# Autodesk Inventor assembly: chassis_2-02
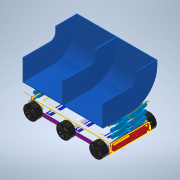
[picture p0: Inventor's stored thumbnail of the model, 180x180]
Saved by Autodesk Inventor 2022 (Build 260153000, 153)
## iProperties
Created: 2023-03-24
Part Number: chassis_2-02
Document SubType Name: Assembly
Designer: Johnny Jou
Author: Johnny Jou
## Documents named in this file (24)
- C:\Users\JOU\Desktop\git\Areo_Rider_Cabin\car\chassis_2.iam
- C:\Users\JOU\Desktop\git\Areo_Rider_Cabin\car\chassis_1_1.ipt
- C:\Users\JOU\Desktop\git\Areo_Rider_Cabin\car\chassis_1_2.ipt
- C:\Users\JOU\Desktop\git\Areo_Rider_Cabin\car\wheel.ipt
- C:\Users\JOU\Desktop\git\Areo_Rider_Cabin\car\wheel_base_cover.ipt
- C:\Users\JOU\Desktop\git\Areo_Rider_Cabin\car\bearing.iam
- C:\Users\JOU\Desktop\git\Areo_Rider_Cabin\car\axle 4_20.ipt
- C:\Users\JOU\Desktop\git\Areo_Rider_Cabin\car\Coupling.ipt
- C:\Users\JOU\Desktop\git\Areo_Rider_Cabin\car\chassis_1_1\chassis_1_1-01.ipt
- C:\Users\JOU\Desktop\git\Areo_Rider_Cabin\Expansion\gasket.ipt
- C:\Users\JOU\Desktop\git\Areo_Rider_Cabin\Expansion\link_2022.ipt
- C:\Users\JOU\Desktop\git\Areo_Rider_Cabin\Expansion\rod_2.ipt
- C:\Users\JOU\Desktop\git\Areo_Rider_Cabin\car\chassis_1_1\chassis_1_1-02.ipt
- C:\Users\JOU\Desktop\git\Areo_Rider_Cabin\car\外抓檔\25GA370.ipt
- C:\Users\JOU\Desktop\git\Areo_Rider_Cabin\Expansion\rod_3.ipt
- C:\Users\JOU\Desktop\git\Areo_Rider_Cabin\car\chassis_1_3.ipt
- C:\Users\JOU\Desktop\git\Areo_Rider_Cabin\car\chassis_1_4.ipt
- C:\Users\JOU\Desktop\git\Areo_Rider_Cabin\car\chassis_1_2_up.ipt
- C:\Users\JOU\Desktop\git\Areo_Rider_Cabin\Airfoil & Nuzzle\nuzzle\nuzzle_v2_0327.ipt
- C:\Users\Johnny Jou\Documents\GitHub\Areo_Rider_Cabin\car\chassis_2\AIP\FEA\eaz3jbjy8.fins
- C:\Users\Johnny Jou\Documents\GitHub\Areo_Rider_Cabin\car\chassis_2\AIP\FEA\eaz3jbjy8.fsat
- C:\Users\Johnny Jou\Documents\GitHub\Areo_Rider_Cabin\car\chassis_2\AIP\FEA\eaz3jbjy8.ftes
- C:\Users\Johnny Jou\Documents\GitHub\Areo_Rider_Cabin\car\chassis_2\AIP\FEA\eaz3jbjy8.fwiz
- C:\Users\Johnny Jou\Documents\GitHub\Areo_Rider_Cabin\car\chassis_2\AIP\FEA\eaz3jbk9s.fmsh
## Components (61 placed, 17 different names)
1. chassis_1_1-02:1 — 貼合:1, 齊平:1, 貼合:2, 齊平:2, 貼合:4, 貼合:5, 貼合:8, 貼合:9, 貼合:10, 貼合:14, 貼合:28, 貼合:29, 貼合:30, 貼合:31, 貼合:39, 貼合:40, 貼合:41, 齊平:12, 貼合:102, 齊平:13, 貼合:103, 貼合:104, 貼合:105, 齊平:14, 貼合:106, 齊平:15, 貼合:110, 貼合:111
2. chassis_1_2:1 — 貼合:1, 齊平:1, 貼合:2, 貼合:62, 角度:1, 相切:2, 貼合:96, 貼合:97, 齊平:17
3. chassis_1_2:2 — 齊平:2, 貼合:4, 貼合:5, 貼合:6, 貼合:7, 齊平:3, 相切:1, 貼合:93, 貼合:95, 貼合:109
4. chassis_1_1-01:2 — 貼合:6, 貼合:7, 齊平:3, 貼合:18, 貼合:19, 貼合:20, 貼合:21, 貼合:56, 貼合:57, 貼合:58, 貼合:59, 貼合:60, 貼合:61, 齊平:11, 貼合:107, 貼合:108
5. 25GA370:1 — 貼合:8, 貼合:9, 貼合:10, 貼合:11
6. Coupling:1 — 貼合:11, 貼合:12, 貼合:13, 貼合:14
7. wheel:1 — 貼合:12, 貼合:13
8. 25GA370:2 — 貼合:18, 貼合:20, 貼合:21
9. Coupling:2 — 貼合:19
10. wheel:2
11. Coupling:3 — 貼合:27, 貼合:28
12. wheel:3
13. 軸承:1 [sub-assembly] — 貼合:24, 貼合:25, 貼合:26, 齊平:4
14. wheel_base_cover:1 — 貼合:24, 貼合:25, 貼合:30, 貼合:31
15. axle 4_20:1 — 貼合:26, 齊平:4, 貼合:27, 貼合:29
16. Coupling:4 — 貼合:38
17. wheel:4
18. 軸承:2 [sub-assembly]
19. wheel_base_cover:2 — 貼合:38, 貼合:39, 貼合:40, 貼合:41
20. axle 4_20:2
21. Coupling:5
22. wheel:5
23. 軸承:3 [sub-assembly]
24. wheel_base_cover:3 — 貼合:56, 貼合:57, 貼合:58
25. axle 4_20:3
26. Coupling:6
27. wheel:6 — 齊平:16
28. 軸承:4 [sub-assembly]
29. wheel_base_cover:4 — 貼合:59, 貼合:60, 貼合:61
30. axle 4_20:4
31. rod_2:1 — 貼合:62, 角度:1, 貼合:63, 貼合:64, 貼合:65, 貼合:66, 貼合:94, 貼合:98
32. 軸承:5 [sub-assembly] — 貼合:63, 貼合:64, 相切:1
33. 軸承:6 [sub-assembly] — 貼合:65, 貼合:66, 相切:2
34. link_2022:1 — 貼合:67, up_and_down, 貼合:70, 貼合:71, 貼合:75, 貼合:94, 插入:3, 齊平:9, 貼合:100
35. link_2022:2 — 貼合:67, up_and_down, 貼合:70, 貼合:76, 貼合:91, 貼合:92, 貼合:93
36. link_2022:3 — 貼合:72, 貼合:76, 貼合:78, 齊平:8, 貼合:99
37. link_2022:4 — 貼合:71, 貼合:72, 貼合:73, 貼合:75, 貼合:77
38. link_2022:5 — 貼合:73, 貼合:74, 貼合:77, 齊平:10, 貼合:101, 插入:6
39. link_2022:6 — 貼合:74, 貼合:78, 貼合:112
40. link_2022:7 — 貼合:96, 貼合:97, 插入:2
41. link_2022:8 — 貼合:98, 插入:1
42. link_2022:9
43. link_2022:10
44. link_2022:11 — 貼合:113
45. link_2022:12 — 插入:4
46. gasket:1 — 貼合:91, 貼合:92, 貼合:95
47. gasket:2 — 插入:1
48. gasket:3 — 插入:2
49. gasket:4 — 插入:3
50. rod_3:1 — 齊平:8, 貼合:99
51. rod_3:2 — 齊平:9, 貼合:100
52. rod_3:3 — 齊平:10, 貼合:101
53. chassis_1_3:1 — 齊平:11, 齊平:12, 貼合:102
54. chassis_1_3:2 — 齊平:15, 貼合:110, 貼合:111
55. chassis_1_3:3 — 齊平:13, 貼合:103, 貼合:104
56. chassis_1_3:4 — 貼合:105, 齊平:14, 貼合:106
57. chassis_1_4:1 — 貼合:107, 貼合:108, 貼合:109
58. chassis_1_2_up:1 — 插入:5, 貼合:112, 貼合:114
59. chassis_1_2_up:2 — 插入:4, 貼合:113
60. gasket:5 — 插入:5, 插入:6
61. nuzzle_v2_0327:1 — 貼合:114, 齊平:16, 齊平:17
## Relationships (145: Mate 113, Flush 17, Angle 7, Insert 6, Tangent 2)
- 貼合:1 [Mate]: chassis_1_1-02:1 ↔ chassis_1_2:1
- 齊平:1 [Flush]: chassis_1_1-02:1 ↔ chassis_1_2:1
- 貼合:2 [Mate]: chassis_1_1-02:1 ↔ chassis_1_2:1
- 齊平:2 [Flush]: chassis_1_1-02:1 ↔ chassis_1_2:2
- 貼合:4 [Mate]: chassis_1_1-02:1 ↔ chassis_1_2:2
- 貼合:5 [Mate]: chassis_1_1-02:1 ↔ chassis_1_2:2
- 貼合:6 [Mate]: chassis_1_2:2 ↔ chassis_1_1-01:2
- 貼合:7 [Mate]: chassis_1_2:2 ↔ chassis_1_1-01:2
- 齊平:3 [Flush]: chassis_1_2:2 ↔ chassis_1_1-01:2
- 貼合:8 [Mate]: chassis_1_1-02:1 ↔ 25GA370:1
- 貼合:9 [Mate]: chassis_1_1-02:1 ↔ 25GA370:1
- 貼合:10 [Mate]: chassis_1_1-02:1 ↔ 25GA370:1
- 貼合:11 [Mate]: 25GA370:1 ↔ Coupling:1
- 貼合:12 [Mate]: Coupling:1 ↔ wheel:1
- 貼合:13 [Mate]: Coupling:1 ↔ wheel:1
- 貼合:14 [Mate] (3 mm): chassis_1_1-02:1 ↔ Coupling:1
- [Mate]: 25GA370:2 ↔ Coupling:2
- [Mate]: Coupling:2 ↔ wheel:2
- [Mate]: Coupling:2 ↔ wheel:2
- 貼合:18 [Mate]: chassis_1_1-01:2 ↔ 25GA370:2
- 貼合:19 [Mate] (3 mm): chassis_1_1-01:2 ↔ Coupling:2
- 貼合:20 [Mate]: chassis_1_1-01:2 ↔ 25GA370:2
- 貼合:21 [Mate]: chassis_1_1-01:2 ↔ 25GA370:2
- [Mate]: Coupling:3 ↔ wheel:3
- [Mate]: Coupling:3 ↔ wheel:3
- 貼合:24 [Mate]: 軸承:1 ↔ wheel_base_cover:1
- 貼合:25 [Mate]: 軸承:1 ↔ wheel_base_cover:1
- 貼合:26 [Mate]: 軸承:1 ↔ axle 4_20:1
- 齊平:4 [Flush]: 軸承:1 ↔ axle 4_20:1
- 貼合:27 [Mate]: Coupling:3 ↔ axle 4_20:1
- 貼合:28 [Mate] (3 mm): chassis_1_1-02:1 ↔ Coupling:3
- 貼合:29 [Mate]: chassis_1_1-02:1 ↔ axle 4_20:1
- 貼合:30 [Mate]: chassis_1_1-02:1 ↔ wheel_base_cover:1
- 貼合:31 [Mate]: chassis_1_1-02:1 ↔ wheel_base_cover:1
- [Mate]: Coupling:4 ↔ wheel:4
- [Mate]: Coupling:4 ↔ wheel:4
- [Mate]: 軸承:2 ↔ wheel_base_cover:2
- [Mate]: 軸承:2 ↔ wheel_base_cover:2
- [Mate]: 軸承:2 ↔ axle 4_20:2
- [Flush]: 軸承:2 ↔ axle 4_20:2
- [Mate]: Coupling:4 ↔ axle 4_20:2
- 貼合:38 [Mate] (6 mm): Coupling:4 ↔ wheel_base_cover:2
- 貼合:39 [Mate]: chassis_1_1-02:1 ↔ wheel_base_cover:2
- 貼合:40 [Mate]: chassis_1_1-02:1 ↔ wheel_base_cover:2
- 貼合:41 [Mate]: chassis_1_1-02:1 ↔ wheel_base_cover:2
- [Mate]: Coupling:5 ↔ wheel:5
- [Mate]: Coupling:5 ↔ wheel:5
- [Mate]: 軸承:3 ↔ wheel_base_cover:3
- [Mate]: 軸承:3 ↔ wheel_base_cover:3
- [Mate]: 軸承:3 ↔ axle 4_20:3
- [Flush]: 軸承:3 ↔ axle 4_20:3
- [Mate]: Coupling:5 ↔ axle 4_20:3
- [Mate] (6 mm): Coupling:5 ↔ wheel_base_cover:3
- [Mate]: Coupling:6 ↔ wheel:6
- [Mate]: Coupling:6 ↔ wheel:6
- [Mate]: 軸承:4 ↔ wheel_base_cover:4
- [Mate]: 軸承:4 ↔ wheel_base_cover:4
- [Mate]: 軸承:4 ↔ axle 4_20:4
- [Flush]: 軸承:4 ↔ axle 4_20:4
- [Mate]: Coupling:6 ↔ axle 4_20:4
- [Mate] (6 mm): Coupling:6 ↔ wheel_base_cover:4
- 貼合:56 [Mate]: chassis_1_1-01:2 ↔ wheel_base_cover:3
- 貼合:57 [Mate]: chassis_1_1-01:2 ↔ wheel_base_cover:3
- 貼合:58 [Mate]: chassis_1_1-01:2 ↔ wheel_base_cover:3
- 貼合:59 [Mate]: chassis_1_1-01:2 ↔ wheel_base_cover:4
- 貼合:60 [Mate]: chassis_1_1-01:2 ↔ wheel_base_cover:4
- 貼合:61 [Mate]: chassis_1_1-01:2 ↔ wheel_base_cover:4
- 貼合:62 [Mate]: chassis_1_2:1 ↔ rod_2:1
- 角度:1 [Angle] (0 deg): chassis_1_2:1 ↔ rod_2:1
- 貼合:63 [Mate]: rod_2:1 ↔ 軸承:5
- 貼合:64 [Mate]: rod_2:1 ↔ 軸承:5
- 貼合:65 [Mate]: rod_2:1 ↔ 軸承:6
- 貼合:66 [Mate]: rod_2:1 ↔ 軸承:6
- 相切:1 [Tangent]: chassis_1_2:2 ↔ 軸承:5
- 相切:2 [Tangent]: chassis_1_2:1 ↔ 軸承:6
- 貼合:67 [Mate]: link_2022:1 ↔ link_2022:2
- up_and_down [Angle] (20 deg): link_2022:1 ↔ link_2022:2
- [Mate]: link_2022:3 ↔ link_2022:4
- [Angle] (20 deg): link_2022:3 ↔ link_2022:4
- [Mate]: link_2022:5 ↔ link_2022:6
- [Angle] (20 deg): link_2022:5 ↔ link_2022:6
- 貼合:70 [Mate]: link_2022:1 ↔ link_2022:2
- 貼合:71 [Mate]: link_2022:1 ↔ link_2022:4
- 貼合:72 [Mate]: link_2022:3 ↔ link_2022:4
- 貼合:73 [Mate]: link_2022:4 ↔ link_2022:5
- 貼合:74 [Mate]: link_2022:5 ↔ link_2022:6
- 貼合:75 [Mate]: link_2022:1 ↔ link_2022:4
- 貼合:76 [Mate]: link_2022:2 ↔ link_2022:3
- 貼合:77 [Mate]: link_2022:4 ↔ link_2022:5
- 貼合:78 [Mate]: link_2022:3 ↔ link_2022:6
- [Mate]: link_2022:7 ↔ link_2022:8
- [Angle] (20 deg): link_2022:7 ↔ link_2022:8
- [Mate]: link_2022:9 ↔ link_2022:10
- [Angle] (20 deg): link_2022:9 ↔ link_2022:10
- [Mate]: link_2022:11 ↔ link_2022:12
- [Angle] (20 deg): link_2022:11 ↔ link_2022:12
- [Mate]: link_2022:7 ↔ link_2022:8
- [Mate]: link_2022:7 ↔ link_2022:10
- [Mate]: link_2022:9 ↔ link_2022:10
- [Mate]: link_2022:10 ↔ link_2022:11
- [Mate]: link_2022:11 ↔ link_2022:12
- [Mate]: link_2022:7 ↔ link_2022:10
- [Mate]: link_2022:8 ↔ link_2022:9
- [Mate]: link_2022:10 ↔ link_2022:11
- [Mate]: link_2022:9 ↔ link_2022:12
- 貼合:91 [Mate]: link_2022:2 ↔ gasket:1
- 貼合:92 [Mate]: link_2022:2 ↔ gasket:1
- 貼合:93 [Mate]: chassis_1_2:2 ↔ link_2022:2
- 貼合:94 [Mate]: rod_2:1 ↔ link_2022:1
- 貼合:95 [Mate]: chassis_1_2:2 ↔ gasket:1
- 貼合:96 [Mate]: chassis_1_2:1 ↔ link_2022:7
- 貼合:97 [Mate]: chassis_1_2:1 ↔ link_2022:7
- 貼合:98 [Mate]: rod_2:1 ↔ link_2022:8
- 插入:1 [Insert]: link_2022:8 ↔ gasket:2
- 插入:2 [Insert]: link_2022:7 ↔ gasket:3
- 插入:3 [Insert]: link_2022:1 ↔ gasket:4
- 齊平:8 [Flush]: link_2022:3 ↔ rod_3:1
- 貼合:99 [Mate]: link_2022:3 ↔ rod_3:1
- 齊平:9 [Flush]: link_2022:1 ↔ rod_3:2
- 貼合:100 [Mate]: link_2022:1 ↔ rod_3:2
- 齊平:10 [Flush]: link_2022:5 ↔ rod_3:3
- 貼合:101 [Mate]: link_2022:5 ↔ rod_3:3
- 齊平:11 [Flush]: chassis_1_1-01:2 ↔ chassis_1_3:1
- 齊平:12 [Flush]: chassis_1_1-02:1 ↔ chassis_1_3:1
- 貼合:102 [Mate]: chassis_1_1-02:1 ↔ chassis_1_3:1
- 齊平:13 [Flush]: chassis_1_1-02:1 ↔ chassis_1_3:3
- 貼合:103 [Mate]: chassis_1_1-02:1 ↔ chassis_1_3:3
- 貼合:104 [Mate]: chassis_1_1-02:1 ↔ chassis_1_3:3
- 貼合:105 [Mate]: chassis_1_1-02:1 ↔ chassis_1_3:4
- 齊平:14 [Flush]: chassis_1_1-02:1 ↔ chassis_1_3:4
- 貼合:106 [Mate]: chassis_1_1-02:1 ↔ chassis_1_3:4
- 貼合:107 [Mate]: chassis_1_1-01:2 ↔ chassis_1_4:1
- 貼合:108 [Mate]: chassis_1_1-01:2 ↔ chassis_1_4:1
- 貼合:109 [Mate]: chassis_1_2:2 ↔ chassis_1_4:1
- 齊平:15 [Flush]: chassis_1_1-02:1 ↔ chassis_1_3:2
- 貼合:110 [Mate]: chassis_1_1-02:1 ↔ chassis_1_3:2
- 貼合:111 [Mate]: chassis_1_1-02:1 ↔ chassis_1_3:2
- 插入:4 [Insert]: link_2022:12 ↔ chassis_1_2_up:2
- 插入:5 [Insert]: chassis_1_2_up:1 ↔ gasket:5
- 插入:6 [Insert]: link_2022:5 ↔ gasket:5
- 貼合:112 [Mate]: link_2022:6 ↔ chassis_1_2_up:1
- 貼合:113 [Mate]: link_2022:11 ↔ chassis_1_2_up:2
- 貼合:114 [Mate]: chassis_1_2_up:1 ↔ nuzzle_v2_0327:1
- 齊平:16 [Flush]: wheel:6 ↔ nuzzle_v2_0327:1
- 齊平:17 [Flush]: chassis_1_2:1 ↔ nuzzle_v2_0327:1
## Named parameters: sa_0 = 137.2, d355_d351 = 0 mm, d356_d352 = 0 mm, d357_d353 = 0 mm, d362_d352 = 0 mm, d363_d353 = 0 mm, d373_d362_d352 = 0 mm, d374_d363_d353 = 0 mm, d375_d364 = 0 mm, d376_d365 = 0 mm, d377_d366 = 0 mm, d378_d367 = 0 mm, d379_d368 = 0 mm, d384_d373_d362_d352 = 0 mm, d385_d374_d363_d353 = 0 mm, d386_d375_d364 = 0 mm, d387_d376_d365 = 0 mm, d388_d377_d366 = 0 mm, d389_d378_d367 = 0 mm, d390_d379_d368 = 0 mm, d391_d380 = 6 mm, d392_d373_d362_d352 = 0 mm, d393_d374_d363_d353 = 0 mm, d394_d375_d364 = 0 mm, d395_d376_d365 = 0 mm, d396_d377_d366 = 0 mm, d397_d378_d367 = 0 mm, d398_d379_d368 = 0 mm, d399_d380 = 6 mm, d416_d414 = 0 mm, d417_d415 = 20 deg, d418_d414 = 0 mm, d419_d415 = 20 deg, d435_d424 = 0 mm, d436_d425 = 0 mm, d437_d426 = 0 mm, d438_d427 = 0 mm, d439_d428 = 0 mm, d440_d414 = 0 mm, d441_d415 = 20 deg, d442_d416_d414 = 0 mm, d444_d418_d414 = 0 mm, d446_d420 = 0 mm, d447_d421 = 0 mm, d448_d422 = 0 mm, d449_d423 = 0 mm
note: some values were not read from the file. Shown as the stored number, unit unknown: "sa_0".
